# Autodesk Inventor assembly: omni
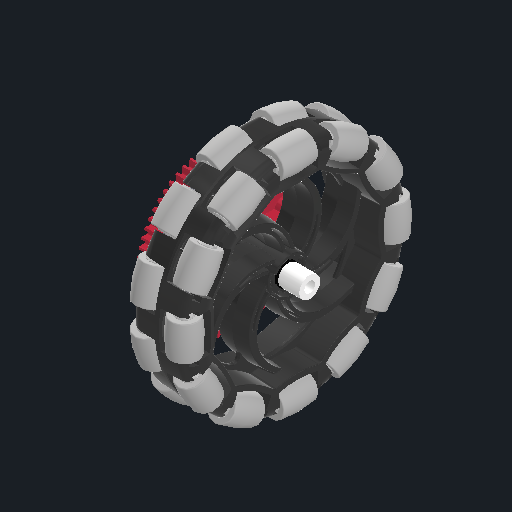
[picture p0: Inventor's stored thumbnail of the model, 512x512]
Saved by Autodesk Inventor 2023 (Build 270158000, 158)
## iProperties
Created: 2023-03-08
Part Number: omni
Document SubType Name: Assembly
Designer: Windows Macbook
Author: Windows Macbook
## Documents named in this file (9)
- C:\Users\Windows Macbook\Desktop\VRC-SPIN-UP\Inventor\Assembly\Pre Worlds\V1\omni.iam
- C:\Users\Windows Macbook\Desktop\VRC-SPIN-UP\Inventor\Motion\Wheels\Omni Wheel\4 Omni, Square.iam
- C:\Users\Windows Macbook\Desktop\VRC-SPIN-UP\Inventor\Motion\Wheels\Omni Wheel.iam
- C:\Users\Windows Macbook\Desktop\VRC-SPIN-UP\Inventor\Motion\Spacers\Spacer Nylon .313 OD\NSpacer .313 OD x .375.ipt
- C:\Users\Windows Macbook\Desktop\VRC-SPIN-UP\Inventor\Motion\Spacers\Spacer Nylon .313 OD.ipt
- C:\Users\Windows Macbook\Desktop\VRC-SPIN-UP\Inventor\Motion\Spacers\Spacer Nylon .313 OD\NSpacer .313 OD x .250.ipt
- C:\Users\Windows Macbook\Desktop\VRC-SPIN-UP\Inventor\Motion\Gears\HS Gear\HS 60T Gear, Square.iam
- C:\Users\Windows Macbook\Desktop\VRC-SPIN-UP\Inventor\Motion\Gears\HS Gear.iam
- C:\Users\Windows Macbook\Desktop\VRC-SPIN-UP\Inventor\Motion\Spacers\Spacer Nylon .313 OD\NSpacer .313 OD x .125.ipt
## Components (5 placed, 5 different names)
1. 4 Omni, Square:1 [sub-assembly]
2. NSpacer .313 OD x .375:1
3. NSpacer .313 OD x .250:2
4. HS 60T Gear, Square:1 [sub-assembly]
5. NSpacer .313 OD x .125:3
## Relationships (4: Insert 4)
- [Insert]: 4 Omni, Square:1 ↔ NSpacer .313 OD x .375:1
- [Insert]: 4 Omni, Square:1 ↔ NSpacer .313 OD x .250:2
- [Insert]: NSpacer .313 OD x .250:2 ↔ HS 60T Gear, Square:1
- [Insert]: HS 60T Gear, Square:1 ↔ NSpacer .313 OD x .125:3
